# Autodesk Inventor assembly: ATLAS ASSEMBLY
(part 2 of 2)
- Mate:352: 98804A029 Long Threaded Rod:1 ↔ 92141A029 0.25 Washer:12
- Mate:353: ODSY-0007-004:2 ↔ 92141A029 0.25 Washer:12
- Mate:354: 98804A029 Long Threaded Rod:1 ↔ 92141A029 0.25 Washer:11
- Mate:355: ODSY-0007-004:2 ↔ 92141A029 0.25 Washer:11
- Mate:356: 98804A029 Long Threaded Rod:1 ↔ 92141A029 0.25 Washer:9
- Mate:357: ODSY-0007-004:1 ↔ 92141A029 0.25 Washer:9
- Mate:358: 98804A029 Long Threaded Rod:1 ↔ 92141A029 0.25 Washer:10
- Mate:359: ODSY-0007-004:1 ↔ 92141A029 0.25 Washer:10
- Mate:360: 98804A029 Long Threaded Rod:2 ↔ 92141A029 0.25 Washer:13
- Mate:361: 98804A029 Long Threaded Rod:2 ↔ 92141A029 0.25 Washer:14
- Mate:362: 98804A029 Long Threaded Rod:2 ↔ 92141A029 0.25 Washer:15
- Mate:363: 98804A029 Long Threaded Rod:2 ↔ 92141A029 0.25 Washer:16
- Mate:364: 98804A029 Long Threaded Rod:2 ↔ 92141A029 0.25 Washer:17
- Mate:365: 98804A029 Long Threaded Rod:2 ↔ 92141A029 0.25 Washer:18
- Mate:366: 98804A029 Long Threaded Rod:1 ↔ 92141A029 0.25 Washer:20
- Mate:367: 98804A029 Long Threaded Rod:1 ↔ 92141A029 0.25 Washer:19
- Mate:368: ODSY-0007-001:1 ↔ 92141A029 0.25 Washer:17
- Mate:369: ODSY-0007-001:1 ↔ 92141A029 0.25 Washer:19
- Mate:370: ODSY-0007-001:1 ↔ 92141A029 0.25 Washer:20
- Mate:371: ODSY-0007-001:1 ↔ 92141A029 0.25 Washer:18
- Mate:372: ODSY-0007-004:2 ↔ 92141A029 0.25 Washer:15
- Mate:373: ODSY-0007-004:2 ↔ 92141A029 0.25 Washer:16
- Mate:374: ODSY-0007-004:1 ↔ 92141A029 0.25 Washer:13
- Mate:375: ODSY-0007-004:1 ↔ 92141A029 0.25 Washer:14
- Mate:376: ODSY-0007-003:2 ↔ 91292A209 Bottom Holder Screw:2
- Mate:377: ODSY-0007-003:1 ↔ 91292A209 Bottom Holder Screw:1
- Mate:378: ODSY-0007-003:1 ↔ 91292A209 Bottom Holder Screw:4
- Mate:379: ODSY-0007-003:2 ↔ 91292A209 Bottom Holder Screw:3
- Mate:380: 91292A209 Bottom Holder Screw:2 ↔ 98689A116 Bottom Holder Washer:2
- Mate:381: 91292A209 Bottom Holder Screw:1 ↔ 98689A116 Bottom Holder Washer:1
- Mate:382: 91292A209 Bottom Holder Screw:4 ↔ 98689A116 Bottom Holder Washer:3
- Mate:383: 91292A209 Bottom Holder Screw:3 ↔ 98689A116 Bottom Holder Washer:4
- Mate:384: ODSY-0007-003:1 ↔ 98689A116 Bottom Holder Washer:3
- Mate:385: ODSY-0007-003:2 ↔ 98689A116 Bottom Holder Washer:4
- Mate:386: ODSY-0007-003:2 ↔ 98689A116 Bottom Holder Washer:2
- Mate:387: ODSY-0007-003:1 ↔ 98689A116 Bottom Holder Washer:1
- Mate:388: 91292A209 Bottom Holder Screw:1 ↔ 98689A116 Bottom Holder Washer:1
- Mate:389: 91292A209 Bottom Holder Screw:2 ↔ 98689A116 Bottom Holder Washer:2
- Mate:390: 91292A209 Bottom Holder Screw:4 ↔ 98689A116 Bottom Holder Washer:3
- Mate:391: 91292A209 Bottom Holder Screw:3 ↔ 98689A116 Bottom Holder Washer:4
- Mate:392: 95412A566 Short Threaded Rod:2 ↔ 91845A029 0.25 Nut:4
- Mate:393: 95412A566 Short Threaded Rod:2 ↔ 91845A029 0.25 Nut:2
- Flush:136: 91845A029 0.25 Nut:2 ↔ 91845A029 0.25 Nut:4
- Mate:394: 92141A029 0.25 Washer:6 ↔ 91845A029 0.25 Nut:4
- Mate:395: 91845A029 0.25 Nut:2 ↔ 91845A029 0.25 Nut:4
- Mate:396: 92141A029 0.25 Washer:8 ↔ 91845A029 0.25 Nut:8
- Mate:397: 95412A566 Short Threaded Rod:4 ↔ 91845A029 0.25 Nut:8
- Mate:398: 95412A566 Short Threaded Rod:4 ↔ 91845A029 0.25 Nut:5
- Flush:137: 91845A029 0.25 Nut:5 ↔ 91845A029 0.25 Nut:8
- Mate:399: 91845A029 0.25 Nut:5 ↔ 91845A029 0.25 Nut:8
- Mate:400: 95412A566 Short Threaded Rod:1 ↔ 91845A029 0.25 Nut:3
- Mate:401: 95412A566 Short Threaded Rod:1 ↔ 91845A029 0.25 Nut:7
- Flush:138: 91845A029 0.25 Nut:3 ↔ 91845A029 0.25 Nut:7
- Mate:402: 91845A029 0.25 Nut:3 ↔ 91845A029 0.25 Nut:7
- Mate:403: 92141A029 0.25 Washer:7 ↔ 91845A029 0.25 Nut:3
- Mate:404: 95412A566 Short Threaded Rod:3 ↔ 91845A029 0.25 Nut:1
- Mate:405: 95412A566 Short Threaded Rod:3 ↔ 91845A029 0.25 Nut:6
- Mate:406: 91845A029 0.25 Nut:1 ↔ 91845A029 0.25 Nut:6
- Mate:407: 92141A029 0.25 Washer:5 ↔ 91845A029 0.25 Nut:6
- Mate:408: 98804A029 Long Threaded Rod:1 ↔ 91845A029 0.25 Nut:15
- Mate:409: 98804A029 Long Threaded Rod:1 ↔ 91845A029 0.25 Nut:16
- Mate:410: 98804A029 Long Threaded Rod:2 ↔ 91845A029 0.25 Nut:13
- Mate:411: 98804A029 Long Threaded Rod:2 ↔ 91845A029 0.25 Nut:14
- Mate:412: 98804A029 Long Threaded Rod:2 ↔ 91845A029 0.25 Nut:12
- Mate:413: 98804A029 Long Threaded Rod:2 ↔ 91845A029 0.25 Nut:11
- Mate:414: 98804A029 Long Threaded Rod:1 ↔ 91845A029 0.25 Nut:10
- Mate:415: 98804A029 Long Threaded Rod:1 ↔ 91845A029 0.25 Nut:9
- Flush:139: 91845A029 0.25 Nut:9 ↔ 91845A029 0.25 Nut:10
- Mate:416: 92141A029 0.25 Washer:10 ↔ 91845A029 0.25 Nut:9
- Mate:417: 91845A029 0.25 Nut:9 ↔ 91845A029 0.25 Nut:10
- Mate:418: 92141A029 0.25 Washer:9 ↔ 91845A029 0.25 Nut:15
- Mate:419: 91845A029 0.25 Nut:15 ↔ 91845A029 0.25 Nut:16
- Flush:140: 91845A029 0.25 Nut:15 ↔ 91845A029 0.25 Nut:16
- Mate:420: 92141A029 0.25 Washer:13 ↔ 91845A029 0.25 Nut:12
- Mate:421: 91845A029 0.25 Nut:11 ↔ 91845A029 0.25 Nut:12
- Flush:141: 91845A029 0.25 Nut:11 ↔ 91845A029 0.25 Nut:12
- Mate:422: 92141A029 0.25 Washer:14 ↔ 91845A029 0.25 Nut:13
- Mate:423: 91845A029 0.25 Nut:13 ↔ 91845A029 0.25 Nut:14
- Flush:142: 91845A029 0.25 Nut:13 ↔ 91845A029 0.25 Nut:14
- Mate:424: 98804A029 Long Threaded Rod:1 ↔ 91845A029 0.25 Nut:17
- Mate:425: 98804A029 Long Threaded Rod:1 ↔ 91845A029 0.25 Nut:18
- Mate:426: 98804A029 Long Threaded Rod:1 ↔ 91845A029 0.25 Nut:19
- Mate:427: 98804A029 Long Threaded Rod:1 ↔ 91845A029 0.25 Nut:20
- Mate:428: 98804A029 Long Threaded Rod:2 ↔ 91845A029 0.25 Nut:22
- Mate:429: 98804A029 Long Threaded Rod:2 ↔ 91845A029 0.25 Nut:21
- Mate:430: 98804A029 Long Threaded Rod:2 ↔ 91845A029 0.25 Nut:24
- Mate:431: 98804A029 Long Threaded Rod:2 ↔ 91845A029 0.25 Nut:23
- Flush:143: 91845A029 0.25 Nut:23 ↔ 91845A029 0.25 Nut:24
- Flush:144: 91845A029 0.25 Nut:21 ↔ 91845A029 0.25 Nut:22
- Flush:145: 91845A029 0.25 Nut:19 ↔ 91845A029 0.25 Nut:20
- Flush:146: 91845A029 0.25 Nut:17 ↔ 91845A029 0.25 Nut:18
- Mate:432: 92141A029 0.25 Washer:12 ↔ 91845A029 0.25 Nut:17
- Mate:433: 91845A029 0.25 Nut:17 ↔ 91845A029 0.25 Nut:18
- Mate:434: 92141A029 0.25 Washer:11 ↔ 91845A029 0.25 Nut:19
- Mate:435: 91845A029 0.25 Nut:19 ↔ 91845A029 0.25 Nut:20
- Mate:436: 92141A029 0.25 Washer:15 ↔ 91845A029 0.25 Nut:22
- Mate:437: 91845A029 0.25 Nut:21 ↔ 91845A029 0.25 Nut:22
- Mate:438: 92141A029 0.25 Washer:16 ↔ 91845A029 0.25 Nut:23
- Mate:439: 91845A029 0.25 Nut:23 ↔ 91845A029 0.25 Nut:24
- Mate:440: 98804A029 Long Threaded Rod:2 ↔ 91845A029 0.25 Nut:29
- Mate:441: 98804A029 Long Threaded Rod:2 ↔ 91845A029 0.25 Nut:30
- Mate:442: 98804A029 Long Threaded Rod:2 ↔ 91845A029 0.25 Nut:31
- Mate:443: 98804A029 Long Threaded Rod:2 ↔ 91845A029 0.25 Nut:32
- Mate:444: 98804A029 Long Threaded Rod:1 ↔ 91845A029 0.25 Nut:26
- Mate:445: 98804A029 Long Threaded Rod:1 ↔ 91845A029 0.25 Nut:25
- Mate:446: 98804A029 Long Threaded Rod:1 ↔ 91845A029 0.25 Nut:28
- Mate:447: 98804A029 Long Threaded Rod:1 ↔ 91845A029 0.25 Nut:27
- Flush:147: 91845A029 0.25 Nut:27 ↔ 91845A029 0.25 Nut:28
- Mate:448: 91845A029 0.25 Nut:27 ↔ 91845A029 0.25 Nut:28
- Mate:449: 92141A029 0.25 Washer:20 ↔ 91845A029 0.25 Nut:27
- Mate:450: 91845A029 0.25 Nut:29 ↔ 91845A029 0.25 Nut:30
- Flush:148: 91845A029 0.25 Nut:29 ↔ 91845A029 0.25 Nut:30
- Mate:451: 92141A029 0.25 Washer:18 ↔ 91845A029 0.25 Nut:29
- Mate:452: 92141A029 0.25 Washer:19 ↔ 91845A029 0.25 Nut:26
- Mate:453: 91845A029 0.25 Nut:25 ↔ 91845A029 0.25 Nut:26
- Mate:454: 91845A029 0.25 Nut:31 ↔ 91845A029 0.25 Nut:32
- Flush:149: 91845A029 0.25 Nut:31 ↔ 91845A029 0.25 Nut:32
- Mate:455: 92141A029 0.25 Washer:17 ↔ 91845A029 0.25 Nut:31
- Flush:150: 98804A029 Long Threaded Rod:1 ↔ 98804A029 Long Threaded Rod:2
- Flush:151 (25.4 mm): 98804A029 Long Threaded Rod:1 ↔ 91845A029 0.25 Nut:16
- Flush:152 (50.8 mm): 98804A029 Long Threaded Rod:1 ↔ 91845A029 0.25 Nut:28
- Mate:456 (279.4 mm): ODSY-0007-003:1 ↔ ODSY-0007-003:2
- Mate:457: 92196A801 Load Cell Bolt:1 ↔ 91845A029 0.25 Nut:35
- Mate:458: 92196A801 Load Cell Bolt:1 ↔ 91845A029 0.25 Nut:36
- Flush:153: 91845A029 0.25 Nut:35 ↔ 91845A029 0.25 Nut:36
- Mate:459: 92141A029 0.25 Washer:3 ↔ 91845A029 0.25 Nut:35
- Mate:460: 91845A029 0.25 Nut:35 ↔ 91845A029 0.25 Nut:36
- Mate:461: 92196A801 Load Cell Bolt:2 ↔ 91845A029 0.25 Nut:33
- Mate:462: 92141A029 0.25 Washer:4 ↔ 91845A029 0.25 Nut:33
- Mate:463: 92196A801 Load Cell Bolt:2 ↔ 91845A029 0.25 Nut:34
- Flush:154: 91845A029 0.25 Nut:33 ↔ 91845A029 0.25 Nut:34
- Mate:464: 91845A029 0.25 Nut:33 ↔ 91845A029 0.25 Nut:34
- Mate:465: 92196A801 Load Cell Bolt:1 ↔ Load Cell:2
- Mate:466: ODSY-0007-001:1 ↔ Load Cell:2
- Mate:467: ODSY-0007-002:1 ↔ 92196A801 Load Cell Bolt:1
- Mate:468: ODSY-0007-002:1 ↔ 92196A801 Load Cell Bolt:2
- Mate:469: ODSY-0007-002:1 ↔ Load Cell:1
- Mate:470: ODSY-0007-002:1 ↔ 92141A029 0.25 Washer:4
- Mate:471: ODSY-0007-004:1 ↔ 98804A029 Long Threaded Rod:1
- Mate:472: ODSY-0007-001:1 ↔ 98804A029 Long Threaded Rod:1
- Mate:473: 95412A566 Short Threaded Rod:1 ↔ 92510A475 Spacer:2
- Mate:474: ODSY-0007-004:2 ↔ 92510A475 Spacer:2
- Mate:475: 95412A566 Short Threaded Rod:2 ↔ 92510A475 Spacer:1
- Mate:476: ODSY-0007-004:1 ↔ 92510A475 Spacer:1
- Mate:477: 95412A566 Short Threaded Rod:4 ↔ 92510A475 Spacer:4
- Mate:478: ODSY-0007-004:1 ↔ 92510A475 Spacer:4
- Mate:479: 95412A566 Short Threaded Rod:3 ↔ 92510A475 Spacer:3
- Mate:480: ODSY-0007-004:2 ↔ 92510A475 Spacer:3
- Mate:481: ODSY-0007-002:1 ↔ 92196A551 Engine Bolts:1
- Mate:482: 92196A551 Engine Bolts:1 ↔ 90945A760 Washers For Engine:1
- Mate:483: 92196A551 Engine Bolts:1 ↔ 90945A760 Washers For Engine:1
- Mate:484: ODSY-0007-002:1 ↔ 90945A760 Washers For Engine:1
- Mate:485: 92196A551 Engine Bolts:1 ↔ 90945A760 Washers For Engine:2
- Mate:486: ODSY-0007-002:1 ↔ 90945A760 Washers For Engine:2
- Mate:487: 92196A551 Engine Bolts:1 ↔ 90945A760 Washers For Engine:3
- Mate:488: Combustion Chamber Assembly:1 ↔ 90945A760 Washers For Engine:2
- Mate:489: Combustion Chamber Assembly:1 ↔ 90945A760 Washers For Engine:3
- Mate:490: 92196A551 Engine Bolts:1 ↔ 91831A029 Lock Nuts For Engine:1
- Mate:491: 90945A760 Washers For Engine:3 ↔ 91831A029 Lock Nuts For Engine:1
- Mate:492: 4080 6ft:1 ↔ 45 Plate:5
- Mate:493: 4080 6ft:2 ↔ 45 Plate:4
- Flush:155: 45 Plate:4 ↔ 45 Plate:5
- Flush:156: 45 Plate:4 ↔ 45 Plate:5
- Mate:494 (-20 mm): 4080 6ft:2 ↔ 45 Plate:4
- Mate:495 (-20 mm): 4080 6ft:2 ↔ 45 Plate:4
- Mate:496: 45 Plate:4 ↔ Tank Uprights:1
- Mate:497: 45 Plate:5 ↔ Tank Uprights:2
- Mate:498 (-20 mm): 45 Plate:4 ↔ Tank Uprights:1
- Mate:499 (-20 mm): 45 Plate:4 ↔ Tank Uprights:1
- Mate:501: 45 Plate:5 ↔ Tank Uprights:2
- Mate:502 (-20 mm): 45 Plate:5 ↔ Tank Uprights:2
- Mate:503 (-20 mm): 45 Plate:5 ↔ Tank Uprights:2
- Mate:506: Tank Uprights:1 ↔ 4040 2.5ft:13
- Flush:159: Tank Uprights:1 ↔ 4040 2.5ft:13
- Mate:507: Tank Uprights:2 ↔ 4040 2.5ft:12
- Flush:160: Tank Uprights:2 ↔ 4040 2.5ft:12
- Mate:508: 4040 2.5ft:12 ↔ Tank Holder:2
- Mate:509: 4040 2.5ft:13 ↔ Tank Holder:1
- Mate:512: 4040 2.5ft:12 ↔ Tank Holder:2
- Mate:513: 4040 2.5ft:13 ↔ Tank Holder:1
- Flush:161: Tank Uprights:1 ↔ 4040 2.5ft:12
- Flush:163: Tank Uprights:1 ↔ Tank Upright Support:2
- Mate:515: Tank Uprights:1 ↔ Tank Upright Support:2
- Flush:164: Tank Uprights:2 ↔ Tank Upright Support:1
- Mate:516: Tank Uprights:2 ↔ Tank Upright Support:1
- Mate:517: Tank Upright Support:1 ↔ 45 splicer:1
- Flush:165: Tank Upright Support:1 ↔ 45 splicer:1
- Flush:166: Tank Upright Support:1 ↔ 45 splicer:1
- Mate:518: 4080 6ft:1 ↔ 45 splicer:1
- Mate:519: Tank Upright Support:2 ↔ 45 splicer:2
- Flush:167: Tank Upright Support:2 ↔ 45 splicer:2
- Flush:168: Tank Upright Support:2 ↔ 45 splicer:2
- Mate:520: 4080 6ft:2 ↔ 45 splicer:2
- Mate:528 (381 mm): Tank Uprights:2 ↔ Tank Holder:1
- Mate:532 (762 mm): 4040 2.5ft:12 ↔ 4040 2.5ft:13
- Mate:533: 4040 angled:2 ↔ 8080 2.5ft:3
- Mate:534: Tank Upright Support:2 ↔ 40-4340:1
- Mate:535: Tank Upright Support:1 ↔ 40-4340:2
- Mate:536 (-20 mm): Tank Uprights:1 ↔ 40-4340:1
- Mate:537 (-20 mm): Tank Uprights:1 ↔ 40-4340:1
- Mate:538 (-20 mm): Tank Upright Support:2 ↔ 40-4340:1
- Mate:539 (-20 mm): Tank Uprights:2 ↔ 40-4340:2
- Mate:540 (-20 mm): Tank Uprights:2 ↔ 40-4340:2
- Mate:541 (-20 mm): Tank Upright Support:1 ↔ 40-4340:2
- Mate:542: Tank Uprights:1 ↔ 45 splicer:4
- Flush:169: Tank Uprights:1 ↔ 45 splicer:4
- Flush:170: Tank Uprights:1 ↔ 45 splicer:4
- Mate:543: Tank Uprights:2 ↔ 45 splicer:3
- Flush:171: Tank Uprights:2 ↔ 45 splicer:3
- Flush:172: Tank Uprights:2 ↔ 45 splicer:3
- Mate:544: 4080 6ft:2 ↔ 45 splicer:4
- Mate:545: 4080 6ft:1 ↔ 45 splicer:3
- Mate:546: Tank Uprights:2 ↔ 4040 2.5ft:14
- Flush:173: Tank Uprights:2 ↔ 4040 2.5ft:14
- Mate:548: 4040 2.5ft:14 ↔ Tank Holder:3
- Flush:174 (20 mm): 4040 2.5ft:14 ↔ Tank Holder:3
- Mate:550: 4040 2.5ft:12 ↔ 4 Hole Bracket:57
- Mate:551: Tank Uprights:2 ↔ 4 Hole Bracket:57
- Flush:175 (2 mm): 4040 2.5ft:12 ↔ 4 Hole Bracket:57
- Mate:552: Tank Uprights:1 ↔ 4 Hole Bracket:58
- Mate:553: 4040 2.5ft:12 ↔ 4 Hole Bracket:58
- Flush:176 (2 mm): Tank Uprights:1 ↔ 4 Hole Bracket:58
- Mate:554: Tank Uprights:2 ↔ 4 Hole Bracket:59
- Mate:555: 4040 2.5ft:13 ↔ 4 Hole Bracket:59
- Flush:177 (2 mm): Tank Uprights:2 ↔ 4 Hole Bracket:59
- Mate:556: Tank Uprights:1 ↔ 4 Hole Bracket:61
- Mate:557: 4040 2.5ft:13 ↔ 4 Hole Bracket:61
- Flush:178 (2 mm): 4040 2.5ft:13 ↔ 4 Hole Bracket:61
- Mate:558: 4040 2.5ft:13 ↔ 4 Hole Bracket:63
- Mate:559: Tank Uprights:2 ↔ 4 Hole Bracket:63
- Flush:179 (2 mm): Tank Uprights:2 ↔ 4 Hole Bracket:63
- Mate:560: 4040 2.5ft:13 ↔ 4 Hole Bracket:62
- Mate:561: Tank Uprights:1 ↔ 4 Hole Bracket:62
- Flush:180 (2 mm): Tank Uprights:1 ↔ 4 Hole Bracket:62
- Mate:562: 4040 2.5ft:14 ↔ 4 Hole Bracket:64
- Mate:563: Tank Uprights:1 ↔ 4 Hole Bracket:64
- Flush:181 (-2 mm): Tank Uprights:1 ↔ 4 Hole Bracket:64
- Mate:564: 4040 2.5ft:14 ↔ 4 Hole Bracket:65
- Mate:565: Tank Uprights:2 ↔ 4 Hole Bracket:65
- Flush:182 (2 mm): Tank Uprights:2 ↔ 4 Hole Bracket:65
- Mate:566: 4040 2.5ft:14 ↔ 4 Hole Bracket:66
- Mate:567: Tank Uprights:1 ↔ 4 Hole Bracket:66
- Flush:183 (2 mm): Tank Uprights:1 ↔ 4 Hole Bracket:66
- Mate:568: 4040 2.5ft:14 ↔ 4 Hole Bracket:60
- Mate:569: Tank Uprights:2 ↔ 4 Hole Bracket:60
- Flush:184 (2 mm): Tank Uprights:2 ↔ 4 Hole Bracket:60
- Mate:570: Tank Uprights:1 ↔ 45 Plate:6
- Mate:571 (-20 mm): Tank Uprights:1 ↔ 45 Plate:6
- Mate:572 (-20 mm): Tank Uprights:1 ↔ 45 Plate:6
- Mate:573 (-20 mm): Tank Uprights:1 ↔ 45 Plate:6
- Mate:574: 4040 2.5ft:12 ↔ 45 Plate:7
- Mate:575 (-20 mm): 4040 2.5ft:12 ↔ 45 Plate:7
- Mate:576 (-20 mm): 4040 2.5ft:12 ↔ 45 Plate:7
- Mate:577 (-20 mm): Tank Uprights:2 ↔ 45 Plate:7
- Mate:578: Tank Uprights:1 ↔ Odyssey Fluids Panel:1
- Mate:579: 45 splicer:4 ↔ Odyssey Fluids Panel:1
- Flush:185: Tank Uprights:1 ↔ Odyssey Fluids Panel:1
- Flush:186: 4040 2.5ft:14 ↔ Odyssey Fluids Panel:1
- Mate:580: Tank Holder:1 ↔ Tank Holder:2
- Mate:581: Tank Holder:1 ↔ Tank Holder:3
- Mate:582: Tank Holder:2 ↔ Weld Assembly:1
- Mate:583: 4080 6ft:2 ↔ 45 Plate:9
- Mate:584: 4080 6ft:1 ↔ 45 Plate:8
- Mate:585 (-20 mm): 4080 6ft:1 ↔ 45 Plate:8
- Mate:586 (-20 mm): 4080 6ft:1 ↔ 45 Plate:8
- Mate:587 (-20 mm): Tank Upright Support:1 ↔ 45 Plate:8
- Mate:588 (-20 mm): 4080 6ft:2 ↔ 45 Plate:9
- Mate:589 (-20 mm): 4080 6ft:2 ↔ 45 Plate:9
- Mate:590 (-20 mm): Tank Upright Support:2 ↔ 45 Plate:9
- Flush:187: 4080 6ft:2 ↔ 45 Plate:9
